# Autodesk Inventor assembly: FrameTestOutsidePlate
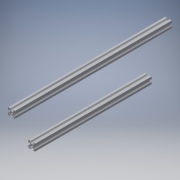
[picture p0: Inventor's stored thumbnail of the model, 180x180]
Saved by Autodesk Inventor 2017 (Build 210142000, 142)
## iProperties
Created: 2018-04-18
Part Number: FrameTestOutsidePlate
Document SubType Name: Assembly
Designer: User
Author: User
## Documents named in this file (3)
- C:\Robotics\CAD\2018-19_CAD\Offseason\FrameTestOutsidePlate.iam
- C:\Robotics\CAD\COTSParts\Bosch Extrusion\Bosch 20x20 17.5 in.ipt
- C:\Robotics\CAD\COTSParts\Bosch Extrusion\Bosch 20x20 13 in - Real.ipt
## Components (2 placed, 2 different names)
1. Bosch 20x20 17.5 in:1 — Flush:1, Flush:2, Mate:1
2. Bosch 20x20 13 in - Real:1 — Flush:1, Flush:2, Mate:1
## Relationships (3: Flush 2, Mate 1)
- Flush:1: Bosch 20x20 17.5 in:1 ↔ Bosch 20x20 13 in - Real:1
- Flush:2 (-57.15 mm): Bosch 20x20 17.5 in:1 ↔ Bosch 20x20 13 in - Real:1
- Mate:1 (88.9 mm): Bosch 20x20 17.5 in:1 ↔ Bosch 20x20 13 in - Real:1
